# Autodesk Inventor assembly: Intake roller assembly
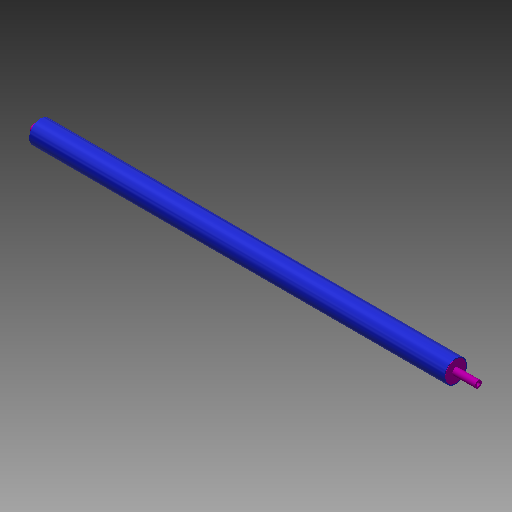
[picture p0: Inventor's stored thumbnail of the model, 512x512]
Saved by Autodesk Inventor 2017 (Build 210142000, 142)
## iProperties
Created: 2017-01-17
Part Number: Intake roller assembly
Document SubType Name: Assembly
Designer: Ben
Author: Ben
## Documents named in this file (4)
- C:\Users\Ben\Desktop\Projects\2017 Robot\Ball Intake\Intake roller assembly.iam
- C:\Users\Ben\Desktop\Projects\2017 Robot\Ball Intake\Intake Roller.ipt
- C:\Users\Ben\Desktop\Projects\2017 Robot\Ball Intake\1in PVC End Cap.ipt
- C:\Users\Ben\Desktop\Projects\2017 Robot\Ball Intake\Long roller plug.ipt
## Components (3 placed, 3 different names)
1. Intake Roller:1 — Insert:1, Insert:2
2. 1in PVC End Cap:1 — Insert:2
3. Long roller plug:1 — Insert:1
## Relationships (2: Insert 2)
- Insert:1: Intake Roller:1 ↔ Long roller plug:1
- Insert:2: Intake Roller:1 ↔ 1in PVC End Cap:1
